# Autodesk Inventor assembly: OurWheelAssembly
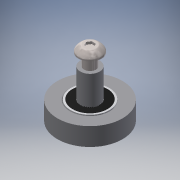
[picture p0: Inventor's stored thumbnail of the model, 180x180]
Saved by Autodesk Inventor 2017 (Build 210142000, 142)
## iProperties
Created: 2017-03-29
Part Number: OurWheelAssembly
Document SubType Name: Assembly
Designer: umr
Author: umr
## Documents named in this file (6)
- D:\SeniorProject\Models2\WheelAssembly\OurWheelAssembly.iam
- D:\SeniorProject\Models2\WheelAssembly\Wheel_16-27.ipt
- D:\SeniorProject\Models2\WheelAssembly\Precision Ball Bearing.ipt
- D:\SeniorProject\Models2\WheelAssembly\M5 Screw_30mm.ipt
- D:\SeniorProject\Models2\WheelAssembly\M5 Nut.ipt
- D:\SeniorProject\Models2\WheelAssembly\egzantrikNut.ipt
## Components (5 placed, 5 different names)
1. Wheel_16-27:1 — Mate:1, Flush:1
2. Precision Ball Bearing:1 — Mate:1, Flush:1, Mate:2, Mate:4, Mate:6
3. M5 Screw_30mm:1 — Mate:2, Mate:3, Mate:5, Mate:7
4. M5 Nut:1 — Mate:3, Mate:4
5. egzantrikNut:2 — Mate:5, Mate:6, Mate:7
## Relationships (8: Mate 7, Flush 1)
- Mate:1: Wheel_16-27:1 ↔ Precision Ball Bearing:1
- Flush:1: Wheel_16-27:1 ↔ Precision Ball Bearing:1
- Mate:2: Precision Ball Bearing:1 ↔ M5 Screw_30mm:1
- Mate:3: M5 Screw_30mm:1 ↔ M5 Nut:1
- Mate:4: Precision Ball Bearing:1 ↔ M5 Nut:1
- Mate:5: M5 Screw_30mm:1 ↔ egzantrikNut:2
- Mate:6: Precision Ball Bearing:1 ↔ egzantrikNut:2
- Mate:7 (5 mm): M5 Screw_30mm:1 ↔ egzantrikNut:2
